# Autodesk Inventor assembly: Assembly_Cube_Mirror_30x30_v3
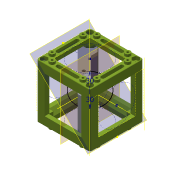
[picture p0: Inventor's stored thumbnail of the model, 180x180]
Saved by Autodesk Inventor 2022 (Build 260153000, 153)
## iProperties
Created: 2020-11-11
Part Number: Assembly_Cube_Mirror_30x30_v3
Document SubType Name: Assembly
Designer: marsikovabarbora
Author: marsikovabarbora
## Documents named in this file (4)
- C:\Users\diederichbenedict\Dropbox\Dokumente\Promotion\PROJECTS\UC2\02_CAD\INVENTOR\uc2_v3\Assembly_Cube_Mirror_Thorlabs_v3.iam
- C:\Users\diederichbenedict\Dropbox\Dokumente\Promotion\PROJECTS\UC2\02_CAD\INVENTOR\uc2_v3\Assembly_Cube_empty_IM_v3.iam
- C:\Users\diederichbenedict\Dropbox\Dokumente\Promotion\PROJECTS\UC2\02_CAD\INVENTOR\uc2_v3\00_Thorlabs_PF10-03-P01-Step.ipt
- C:\Users\diederichbenedict\Dropbox\Dokumente\Promotion\PROJECTS\UC2\02_CAD\INVENTOR\uc2_v3\20_Cube_Insert_Mirror_Holder_Thorlabs_v3.ipt
## Components (3 placed, 3 different names)
1. Assembly_Cube_empty_IM_v3:1 [sub-assembly] — Mate:1, Mate:2, Mate:3, Mate:4, Flush:1, Mate:7, Mate:8
2. 20_Cube_Insert_Mirror_Holder_Thorlabs_v3:1 — Mate:4, Flush:1, Mate:7, Flush:2
3. 00_Thorlabs_PF10-03-P01-Step:1 — Mate:8, Flush:2
## Relationships (8: Mate 6, Flush 2)
- Mate:1: Assembly_Cube_empty_IM_v3:1
- Mate:2: Assembly_Cube_empty_IM_v3:1
- Mate:3: Assembly_Cube_empty_IM_v3:1
- Mate:4: Assembly_Cube_empty_IM_v3:1 ↔ 20_Cube_Insert_Mirror_Holder_Thorlabs_v3:1
- Flush:1 (10 mm): Assembly_Cube_empty_IM_v3:1 ↔ 20_Cube_Insert_Mirror_Holder_Thorlabs_v3:1
- Mate:7: Assembly_Cube_empty_IM_v3:1 ↔ 20_Cube_Insert_Mirror_Holder_Thorlabs_v3:1
- Mate:8: Assembly_Cube_empty_IM_v3:1 ↔ 00_Thorlabs_PF10-03-P01-Step:1
- Flush:2 (-1.5 mm): 20_Cube_Insert_Mirror_Holder_Thorlabs_v3:1 ↔ 00_Thorlabs_PF10-03-P01-Step:1
